# Autodesk Inventor assembly: Mid Flap System Assembly
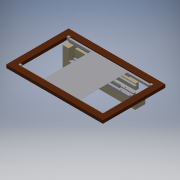
[picture p0: Inventor's stored thumbnail of the model, 180x180]
Saved by Autodesk Inventor 2016 (Build 200138000, 138)
## iProperties
Created: 2016-04-04
Part Number: Mid Flap System Assembly
Document SubType Name: Assembly
Designer: amycroft3
Author: amycroft3
## Documents named in this file (3)
- C:\Users\Ariana\Downloads\Capstone CAD\Capstone CAD\Mid Flap System Assembly.iam
- C:\Users\Ariana\Downloads\Capstone CAD\Capstone CAD\Mid Flaps and Guide Rail Assembly.iam
- C:\Users\Ariana\Downloads\Capstone CAD\Capstone CAD\Rack and Pinion System.iam
## Components (2 placed, 2 different names)
1. Mid Flaps and Guide Rail Assembly:1 [sub-assembly] — Flush:1, Flush:2, Mate:2
2. Rack and Pinion System:1 [sub-assembly] — Flush:1, Flush:2, Mate:2
## Relationships (3: Flush 2, Mate 1)
- Flush:1: Mid Flaps and Guide Rail Assembly:1 ↔ Rack and Pinion System:1
- Flush:2: Mid Flaps and Guide Rail Assembly:1 ↔ Rack and Pinion System:1
- Mate:2: Mid Flaps and Guide Rail Assembly:1 ↔ Rack and Pinion System:1
